# Autodesk Inventor assembly: SpiritBot V1.0
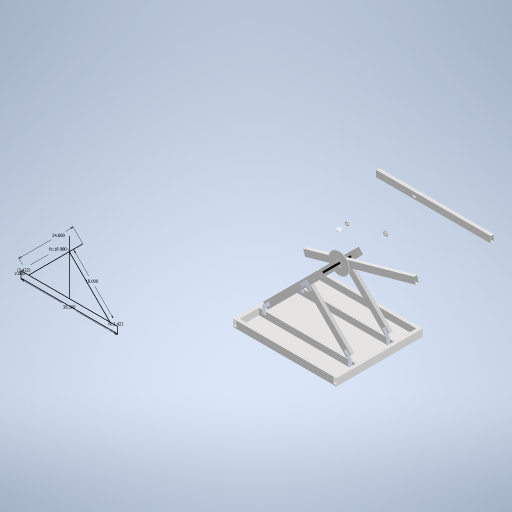
[picture p0: Inventor's stored thumbnail of the model, 512x512]
Saved by Autodesk Inventor 2024 (Build 280153000, 153)
## iProperties
Created: 2023-07-06
Part Number: SpiritBot V1.0
Document SubType Name: Assembly
Designer: Gabriel Marquez
Author: Gabriel Marquez
## Documents named in this file (15)
- C:\Users\Gabriel Marquez\OneDrive\Documents\GitHub\T3-CAD\Current Season CAD\SpiritBot V1.0.iam
- C:\Users\Gabriel Marquez\OneDrive\Documents\GitHub\T3-CAD\Current Season CAD\Body\Base.ipt
- C:\Users\Gabriel Marquez\OneDrive\Documents\GitHub\T3-CAD\Current Season CAD\Body\Long bar 3- VersaFrame.ipt
- C:\Users\Gabriel Marquez\OneDrive\Documents\GitHub\T3-CAD\Current Season CAD\Body\Long bar 4- VersaFrame.ipt
- C:\Users\Gabriel Marquez\OneDrive\Documents\GitHub\T3-CAD\Current Season CAD\Body\Long bar 8.5 - VersaFrame.ipt
- C:\Users\Gabriel Marquez\OneDrive\Documents\GitHub\T3-CAD\Current Season CAD\Body\Long bar 32.3 - VersaFrame.ipt
- C:\Users\Gabriel Marquez\OneDrive\Documents\GitHub\T3-CAD\Stock\Versa System\Gussets\135 Degree Gusset.ipt
- C:\Users\Gabriel Marquez\OneDrive\Documents\GitHub\T3-CAD\Current Season CAD\Body\Super Structure ThunderHex.ipt
- C:\Users\Gabriel Marquez\OneDrive\Documents\GitHub\T3-CAD\Stock\Belts-Chain\Chain\#35\Sprockets\12 Tooth Single.ipt
- C:\Users\Gabriel Marquez\OneDrive\Documents\GitHub\T3-CAD\Stock\Belts-Chain\Chain\#35\Sprockets\54 Tooth plate sprocket.ipt
- C:\Users\Gabriel Marquez\OneDrive\Documents\GitHub\T3-CAD\Current Season CAD\Body\gun turret main spar.ipt
- C:\Users\Gabriel Marquez\OneDrive\Documents\GitHub\T3-CAD\Current Season CAD\Body\Part1.ipt
- C:\Users\Gabriel Marquez\OneDrive\Documents\GitHub\T3-CAD\Stock\Versa System\Gussets\90 Degree Gusset.ipt
- C:\Users\Gabriel Marquez\OneDrive\Documents\GitHub\T3-CAD\Stock\ThunderHex\Shaft Collar.ipt
- C:\Users\Gabriel Marquez\OneDrive\Documents\GitHub\T3-CAD\Stock\ThunderHex\Flanged Bearing.ipt
## Components (25 placed, 14 different names)
1. Base:1 — Mate:7, Mate:8
2. Long bar 32.3 - VersaFrame:1 — Mate:1, Mate:2, Mate:6, Mate:7, Mate:14
3. Long bar 32.3 - VersaFrame:2 — Mate:5, Mate:35
4. Long bar 32.3 - VersaFrame:3 — Mate:10, Mate:11, Mate:14, Rotational:7, Rotational:8
5. Long bar 8.5 - VersaFrame:1 — Mate:1, Mate:2, Mate:5, Mate:11, Mate:34
6. Long bar 8.5 - VersaFrame:2 — Mate:6, Mate:8, Mate:10, Mate:33
7. Super Structure ThunderHex:1 — Cylindrical:1, Mate:36, Cylindrical:2
8. 12 Tooth Single:1
9. 54 Tooth plate sprocket:1 — Cylindrical:2, Mate:37
10. gun turret main spar:1 — Cylindrical:3, Mate:37
11. gun turret main spar:2
12. Long bar 3- VersaFrame:1 — Mate:27, Mate:28, Mate:29, Rotational:1, Rotational:2, Rotational:9, Rotational:10, Cylindrical:1, Mate:36
13. Long bar 4- VersaFrame:2 — Mate:27, Mate:28, Mate:29, Rotational:5, Rotational:6
14. 135 Degree Gusset:13 — Rotational:5, Rotational:6, Rotational:7, Rotational:8
15. Part1:1
16. 90 Degree Gusset:1 — Rotational:1, Rotational:2
17. 135 Degree Gusset:14 — Rotational:9, Rotational:10
18. Long bar 32.3 - VersaFrame:4 — Mate:33, Mate:34, Mate:35
19. Long bar 3- VersaFrame:2 — Cylindrical:3
20. Long bar 4- VersaFrame:3
21. 135 Degree Gusset:15
22. 90 Degree Gusset:2
23. 135 Degree Gusset:16
24. Shaft Collar:1
25. Flanged Bearing:1
## Relationships (41: Mate 22, RevoluteJoint 16, CylindricalJoint 3)
- Mate:1: Long bar 32.3 - VersaFrame:1 ↔ Long bar 8.5 - VersaFrame:1
- Mate:2: Long bar 32.3 - VersaFrame:1 ↔ Long bar 8.5 - VersaFrame:1
- [Mate]: Long bar 32.3 - VersaFrame:2 ↔ Long bar 8.5 - VersaFrame:2
- [Mate]: Long bar 32.3 - VersaFrame:2 ↔ Long bar 8.5 - VersaFrame:2
- Mate:5: Long bar 32.3 - VersaFrame:2 ↔ Long bar 8.5 - VersaFrame:1
- Mate:6: Long bar 32.3 - VersaFrame:1 ↔ Long bar 8.5 - VersaFrame:2
- Mate:7: Base:1 ↔ Long bar 32.3 - VersaFrame:1
- Mate:8: Base:1 ↔ Long bar 8.5 - VersaFrame:2
- Mate:10: Long bar 32.3 - VersaFrame:3 ↔ Long bar 8.5 - VersaFrame:2
- Mate:11: Long bar 32.3 - VersaFrame:3 ↔ Long bar 8.5 - VersaFrame:1
- Mate:14 (152.4 mm): Long bar 32.3 - VersaFrame:1 ↔ Long bar 32.3 - VersaFrame:3
- Mate:27: Long bar 3- VersaFrame:1 ↔ Long bar 4- VersaFrame:2
- Mate:28: Long bar 3- VersaFrame:1 ↔ Long bar 4- VersaFrame:2
- Mate:29 (431.8 mm): Long bar 3- VersaFrame:1 ↔ Long bar 4- VersaFrame:2
- Rotational:1 [RevoluteJoint]: Long bar 3- VersaFrame:1 ↔ 90 Degree Gusset:1
- Rotational:2 [RevoluteJoint]: Long bar 3- VersaFrame:1 ↔ 90 Degree Gusset:1
- Rotational:5 [RevoluteJoint]: Long bar 4- VersaFrame:2 ↔ 135 Degree Gusset:13
- Rotational:6 [RevoluteJoint]: Long bar 4- VersaFrame:2 ↔ 135 Degree Gusset:13
- Rotational:7 [RevoluteJoint]: Long bar 32.3 - VersaFrame:3 ↔ 135 Degree Gusset:13
- Rotational:8 [RevoluteJoint]: Long bar 32.3 - VersaFrame:3 ↔ 135 Degree Gusset:13
- Rotational:9 [RevoluteJoint]: Long bar 3- VersaFrame:1 ↔ 135 Degree Gusset:14
- Rotational:10 [RevoluteJoint]: Long bar 3- VersaFrame:1 ↔ 135 Degree Gusset:14
- [Mate]: Long bar 3- VersaFrame:2 ↔ Long bar 4- VersaFrame:3
- [Mate]: Long bar 3- VersaFrame:2 ↔ Long bar 4- VersaFrame:3
- [Mate] (431.8 mm): Long bar 3- VersaFrame:2 ↔ Long bar 4- VersaFrame:3
- [RevoluteJoint]: Long bar 3- VersaFrame:2 ↔ 90 Degree Gusset:2
- [RevoluteJoint]: Long bar 3- VersaFrame:2 ↔ 90 Degree Gusset:2
- [RevoluteJoint]: Long bar 4- VersaFrame:3 ↔ 135 Degree Gusset:15
- [RevoluteJoint]: Long bar 4- VersaFrame:3 ↔ 135 Degree Gusset:15
- [RevoluteJoint]: Long bar 32.3 - VersaFrame:4 ↔ 135 Degree Gusset:15
- [RevoluteJoint]: Long bar 32.3 - VersaFrame:4 ↔ 135 Degree Gusset:15
- [RevoluteJoint]: Long bar 3- VersaFrame:2 ↔ 135 Degree Gusset:16
- [RevoluteJoint]: Long bar 3- VersaFrame:2 ↔ 135 Degree Gusset:16
- Mate:33: Long bar 8.5 - VersaFrame:2 ↔ Long bar 32.3 - VersaFrame:4
- Mate:34: Long bar 8.5 - VersaFrame:1 ↔ Long bar 32.3 - VersaFrame:4
- Mate:35 (152.4 mm): Long bar 32.3 - VersaFrame:2 ↔ Long bar 32.3 - VersaFrame:4
- Cylindrical:1: Super Structure ThunderHex:1 ↔ Long bar 3- VersaFrame:1
- Mate:36 (38.1 mm): Super Structure ThunderHex:1 ↔ Long bar 3- VersaFrame:1
- Cylindrical:2: Super Structure ThunderHex:1 ↔ 54 Tooth plate sprocket:1
- Cylindrical:3: gun turret main spar:1 ↔ Long bar 3- VersaFrame:2
- Mate:37 (12.7 mm): 54 Tooth plate sprocket:1 ↔ gun turret main spar:1
## Named parameters: d2_d0 = 0 mm, d3_d1 = 0 mm, d155_d128 = 0 mm, d156_d129 = 90 deg, d157_d130 = 0 mm, d158_d131 = 0 deg, d159_d132 = 0 mm, d160_d133 = 45 deg, d161_d134 = 0 mm, d162_d135 = -45 deg, d163_d136 = 0 mm, d164_d137 = -45 deg, d165_d138 = 0 mm, d166_d139 = -45 deg, d167_d114 = 0 mm, d168_d115 = 0 mm, d169_d116 = 431.8 mm, d170_d117 = 0 mm, d171_d118 = 135 deg, d172_d119 = 0 mm, d173_d120 = -135 deg
